# Autodesk Inventor assembly: panelScrewNut
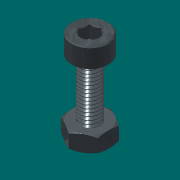
[picture p0: Inventor's stored thumbnail of the model, 180x180]
Saved by Autodesk Inventor 2016 (Build 200138000, 138)
## iProperties
Created: 2015-10-05
Part Number: panelScrewNut
Document SubType Name: Assembly
Designer: Sawaiz
Author: Sawaiz
## Documents named in this file (4)
- C:\Users\sawai\OneDrive\projects\splitFlapDisplay\frame\panelScrewNut.iam
- C:\Users\sawai\OneDrive\projects\splitFlapDisplay\frame\panelNut.ipt
- C:\Users\sawai\OneDrive\projects\splitFlapDisplay\frame\panelScrew.ipt
- C:\Users\sawai\OneDrive\projects\splitFlapDisplay\parameters.xlsx
## Components (2 placed, 2 different names)
1. panelNut:1 — Rotational:1
2. panelScrew:1 — Rotational:1
## Relationships (1: RevoluteJoint 1)
- Rotational:1 [RevoluteJoint] (8.35 mm): panelNut:1 ↔ panelScrew:1
## Named parameters: height = 180 mm, width = 120 mm, depth = 115 mm, materialThickness = 6.35 mm, laserKerf = 0.1 mm, spoolDiameter = 95 mm, cardPinDiameter = 3 mm, cardNumber = 40, centeralShaftDiameter = 8 mm, cardWidth = 85.6 mm, cardHeight = 53.98 mm, cardThickness = 0.76 mm, cardFillet = 2.88 mm, cardCutoutHeight = 20 mm, cardClearence = 0.5 mm, spoolHubDiameter = 20 mm, bearingOd = 22 mm, bearingWidth = 8 mm, axleHeight = 95 mm, nutTrapClearence = 2 mm, nutTrapDepth = 2.5 mm, nutTrapwidth = 5.5 mm, beltLength = 350 mm, magnetLength = 10 mm, magnetDiameter = 6 mm, magnetProtusion = 0.25 mm
